# Autodesk Inventor assembly: HDR_2.54mm_RGB4078660
(part 2 of 3)
- D:\Github\Pandoras_Box\CAD\pandoras_box_R2\pandoras_box_R2\Open CASCADE STEP translator 6.8 1.452.1.450.ipt
- D:\Github\Pandoras_Box\CAD\pandoras_box_R2\pandoras_box_R2\Open CASCADE STEP translator 6.8 1.452.1.451.ipt
- D:\Github\Pandoras_Box\CAD\pandoras_box_R2\pandoras_box_R2\Open CASCADE STEP translator 6.8 1.452.1.452.ipt
- D:\Github\Pandoras_Box\CAD\pandoras_box_R2\pandoras_box_R2\Open CASCADE STEP translator 6.8 1.452.1.453.ipt
- D:\Github\Pandoras_Box\CAD\pandoras_box_R2\pandoras_box_R2\Open CASCADE STEP translator 6.8 1.452.1.454.ipt
- D:\Github\Pandoras_Box\CAD\pandoras_box_R2\pandoras_box_R2\Open CASCADE STEP translator 6.8 1.452.1.455.ipt
- D:\Github\Pandoras_Box\CAD\pandoras_box_R2\pandoras_box_R2\Open CASCADE STEP translator 6.8 1.452.1.456.ipt
- D:\Github\Pandoras_Box\CAD\pandoras_box_R2\pandoras_box_R2\Open CASCADE STEP translator 6.8 1.452.1.457.ipt
- D:\Github\Pandoras_Box\CAD\pandoras_box_R2\pandoras_box_R2\Open CASCADE STEP translator 6.8 1.452.1.458.ipt
- D:\Github\Pandoras_Box\CAD\pandoras_box_R2\pandoras_box_R2\Open CASCADE STEP translator 6.8 1.452.1.459.ipt
- D:\Github\Pandoras_Box\CAD\pandoras_box_R2\pandoras_box_R2\Open CASCADE STEP translator 6.8 1.452.1.460.ipt
- D:\Github\Pandoras_Box\CAD\pandoras_box_R2\pandoras_box_R2\Open CASCADE STEP translator 6.8 1.452.1.461.ipt
- D:\Github\Pandoras_Box\CAD\pandoras_box_R2\pandoras_box_R2\Open CASCADE STEP translator 6.8 1.452.1.462.ipt
- D:\Github\Pandoras_Box\CAD\pandoras_box_R2\pandoras_box_R2\Open CASCADE STEP translator 6.8 1.452.1.463.ipt
- D:\Github\Pandoras_Box\CAD\pandoras_box_R2\pandoras_box_R2\Open CASCADE STEP translator 6.8 1.452.1.464.ipt
- D:\Github\Pandoras_Box\CAD\pandoras_box_R2\pandoras_box_R2\Open CASCADE STEP translator 6.8 1.452.1.465.ipt
- D:\Github\Pandoras_Box\CAD\pandoras_box_R2\pandoras_box_R2\Open CASCADE STEP translator 6.8 1.452.1.466.ipt
- D:\Github\Pandoras_Box\CAD\pandoras_box_R2\pandoras_box_R2\Open CASCADE STEP translator 6.8 1.452.1.467.ipt
- D:\Github\Pandoras_Box\CAD\pandoras_box_R2\pandoras_box_R2\Open CASCADE STEP translator 6.8 1.452.1.468.ipt
- D:\Github\Pandoras_Box\CAD\pandoras_box_R2\pandoras_box_R2\Open CASCADE STEP translator 6.8 1.452.1.469.ipt
- D:\Github\Pandoras_Box\CAD\pandoras_box_R2\pandoras_box_R2\Open CASCADE STEP translator 6.8 1.452.1.470.ipt
- D:\Github\Pandoras_Box\CAD\pandoras_box_R2\pandoras_box_R2\Open CASCADE STEP translator 6.8 1.452.1.471.ipt
- D:\Github\Pandoras_Box\CAD\pandoras_box_R2\pandoras_box_R2\Open CASCADE STEP translator 6.8 1.452.1.472.ipt
- D:\Github\Pandoras_Box\CAD\pandoras_box_R2\pandoras_box_R2\Open CASCADE STEP translator 6.8 1.452.1.473.ipt
- D:\Github\Pandoras_Box\CAD\pandoras_box_R2\pandoras_box_R2\Open CASCADE STEP translator 6.8 1.452.1.474.ipt
- D:\Github\Pandoras_Box\CAD\pandoras_box_R2\pandoras_box_R2\Open CASCADE STEP translator 6.8 1.452.1.475.ipt
- D:\Github\Pandoras_Box\CAD\pandoras_box_R2\pandoras_box_R2\Open CASCADE STEP translator 6.8 1.452.1.476.ipt
- D:\Github\Pandoras_Box\CAD\pandoras_box_R2\pandoras_box_R2\Open CASCADE STEP translator 6.8 1.452.1.477.ipt
- D:\Github\Pandoras_Box\CAD\pandoras_box_R2\pandoras_box_R2\Open CASCADE STEP translator 6.8 1.452.1.478.ipt
- D:\Github\Pandoras_Box\CAD\pandoras_box_R2\pandoras_box_R2\Open CASCADE STEP translator 6.8 1.452.1.479.ipt
- D:\Github\Pandoras_Box\CAD\pandoras_box_R2\pandoras_box_R2\Open CASCADE STEP translator 6.8 1.452.1.480.ipt
- D:\Github\Pandoras_Box\CAD\pandoras_box_R2\pandoras_box_R2\Open CASCADE STEP translator 6.8 1.452.1.481.ipt
- D:\Github\Pandoras_Box\CAD\pandoras_box_R2\pandoras_box_R2\Open CASCADE STEP translator 6.8 1.452.1.482.ipt
- D:\Github\Pandoras_Box\CAD\pandoras_box_R2\pandoras_box_R2\Open CASCADE STEP translator 6.8 1.452.1.483.ipt
- D:\Github\Pandoras_Box\CAD\pandoras_box_R2\pandoras_box_R2\Open CASCADE STEP translator 6.8 1.452.1.484.ipt
- D:\Github\Pandoras_Box\CAD\pandoras_box_R2\pandoras_box_R2\Open CASCADE STEP translator 6.8 1.452.1.485.ipt
- D:\Github\Pandoras_Box\CAD\pandoras_box_R2\pandoras_box_R2\Open CASCADE STEP translator 6.8 1.452.1.486.ipt
- D:\Github\Pandoras_Box\CAD\pandoras_box_R2\pandoras_box_R2\Open CASCADE STEP translator 6.8 1.452.1.487.ipt
- D:\Github\Pandoras_Box\CAD\pandoras_box_R2\pandoras_box_R2\Open CASCADE STEP translator 6.8 1.452.1.488.ipt
- D:\Github\Pandoras_Box\CAD\pandoras_box_R2\pandoras_box_R2\Open CASCADE STEP translator 6.8 1.452.1.489.ipt
- D:\Github\Pandoras_Box\CAD\pandoras_box_R2\pandoras_box_R2\Open CASCADE STEP translator 6.8 1.452.1.490.ipt
- D:\Github\Pandoras_Box\CAD\pandoras_box_R2\pandoras_box_R2\Open CASCADE STEP translator 6.8 1.452.1.491.ipt
- D:\Github\Pandoras_Box\CAD\pandoras_box_R2\pandoras_box_R2\Open CASCADE STEP translator 6.8 1.452.1.492.ipt
- D:\Github\Pandoras_Box\CAD\pandoras_box_R2\pandoras_box_R2\Open CASCADE STEP translator 6.8 1.452.1.493.ipt
- D:\Github\Pandoras_Box\CAD\pandoras_box_R2\pandoras_box_R2\Open CASCADE STEP translator 6.8 1.452.1.494.ipt
- D:\Github\Pandoras_Box\CAD\pandoras_box_R2\pandoras_box_R2\Open CASCADE STEP translator 6.8 1.452.1.495.ipt
- D:\Github\Pandoras_Box\CAD\pandoras_box_R2\pandoras_box_R2\Open CASCADE STEP translator 6.8 1.452.1.496.ipt
- D:\Github\Pandoras_Box\CAD\pandoras_box_R2\pandoras_box_R2\Open CASCADE STEP translator 6.8 1.452.1.497.ipt
- D:\Github\Pandoras_Box\CAD\pandoras_box_R2\pandoras_box_R2\Open CASCADE STEP translator 6.8 1.452.1.498.ipt
- D:\Github\Pandoras_Box\CAD\pandoras_box_R2\pandoras_box_R2\Open CASCADE STEP translator 6.8 1.452.1.499.ipt
- D:\Github\Pandoras_Box\CAD\pandoras_box_R2\pandoras_box_R2\Open CASCADE STEP translator 6.8 1.452.1.500.ipt
- D:\Github\Pandoras_Box\CAD\pandoras_box_R2\pandoras_box_R2\Open CASCADE STEP translator 6.8 1.452.1.501.ipt
- D:\Github\Pandoras_Box\CAD\pandoras_box_R2\pandoras_box_R2\Open CASCADE STEP translator 6.8 1.452.1.502.ipt
- D:\Github\Pandoras_Box\CAD\pandoras_box_R2\pandoras_box_R2\Open CASCADE STEP translator 6.8 1.452.1.503.ipt
- D:\Github\Pandoras_Box\CAD\pandoras_box_R2\pandoras_box_R2\Open CASCADE STEP translator 6.8 1.452.1.504.ipt
- D:\Github\Pandoras_Box\CAD\pandoras_box_R2\pandoras_box_R2\Open CASCADE STEP translator 6.8 1.452.1.505.ipt
- D:\Github\Pandoras_Box\CAD\pandoras_box_R2\pandoras_box_R2\Open CASCADE STEP translator 6.8 1.452.1.506.ipt
- D:\Github\Pandoras_Box\CAD\pandoras_box_R2\pandoras_box_R2\Open CASCADE STEP translator 6.8 1.452.1.507.ipt
- D:\Github\Pandoras_Box\CAD\pandoras_box_R2\pandoras_box_R2\Open CASCADE STEP translator 6.8 1.452.1.508.ipt
- D:\Github\Pandoras_Box\CAD\pandoras_box_R2\pandoras_box_R2\Open CASCADE STEP translator 6.8 1.452.1.509.ipt
- D:\Github\Pandoras_Box\CAD\pandoras_box_R2\pandoras_box_R2\Open CASCADE STEP translator 6.8 1.452.1.510.ipt
- D:\Github\Pandoras_Box\CAD\pandoras_box_R2\pandoras_box_R2\Open CASCADE STEP translator 6.8 1.452.1.511.ipt
- D:\Github\Pandoras_Box\CAD\pandoras_box_R2\pandoras_box_R2\Open CASCADE STEP translator 6.8 1.452.1.512.ipt
- D:\Github\Pandoras_Box\CAD\pandoras_box_R2\pandoras_box_R2\Open CASCADE STEP translator 6.8 1.452.1.513.ipt
- D:\Github\Pandoras_Box\CAD\pandoras_box_R2\pandoras_box_R2\Open CASCADE STEP translator 6.8 1.452.1.514.ipt
- D:\Github\Pandoras_Box\CAD\pandoras_box_R2\pandoras_box_R2\Open CASCADE STEP translator 6.8 1.452.1.515.ipt
- D:\Github\Pandoras_Box\CAD\pandoras_box_R2\pandoras_box_R2\Open CASCADE STEP translator 6.8 1.452.1.516.ipt
- D:\Github\Pandoras_Box\CAD\pandoras_box_R2\pandoras_box_R2\Open CASCADE STEP translator 6.8 1.452.1.517.ipt
- D:\Github\Pandoras_Box\CAD\pandoras_box_R2\pandoras_box_R2\Open CASCADE STEP translator 6.8 1.452.1.518.ipt
- D:\Github\Pandoras_Box\CAD\pandoras_box_R2\pandoras_box_R2\Open CASCADE STEP translator 6.8 1.452.1.519.ipt
- D:\Github\Pandoras_Box\CAD\pandoras_box_R2\pandoras_box_R2\Open CASCADE STEP translator 6.8 1.452.1.520.ipt
- D:\Github\Pandoras_Box\CAD\pandoras_box_R2\pandoras_box_R2\Open CASCADE STEP translator 6.8 1.452.1.521.ipt
- D:\Github\Pandoras_Box\CAD\pandoras_box_R2\pandoras_box_R2\Open CASCADE STEP translator 6.8 1.452.1.522.ipt
- D:\Github\Pandoras_Box\CAD\pandoras_box_R2\pandoras_box_R2\Open CASCADE STEP translator 6.8 1.452.1.523.ipt
- D:\Github\Pandoras_Box\CAD\pandoras_box_R2\pandoras_box_R2\Open CASCADE STEP translator 6.8 1.452.1.524.ipt
- D:\Github\Pandoras_Box\CAD\pandoras_box_R2\pandoras_box_R2\Open CASCADE STEP translator 6.8 1.452.1.525.ipt
- D:\Github\Pandoras_Box\CAD\pandoras_box_R2\pandoras_box_R2\Open CASCADE STEP translator 6.8 1.452.1.526.ipt
- D:\Github\Pandoras_Box\CAD\pandoras_box_R2\pandoras_box_R2\Open CASCADE STEP translator 6.8 1.452.1.527.ipt
- D:\Github\Pandoras_Box\CAD\pandoras_box_R2\pandoras_box_R2\Open CASCADE STEP translator 6.8 1.452.1.528.ipt
- D:\Github\Pandoras_Box\CAD\pandoras_box_R2\pandoras_box_R2\Open CASCADE STEP translator 6.8 1.452.1.529.ipt
- D:\Github\Pandoras_Box\CAD\pandoras_box_R2\pandoras_box_R2\Open CASCADE STEP translator 6.8 1.452.1.530.ipt
- D:\Github\Pandoras_Box\CAD\pandoras_box_R2\pandoras_box_R2\Open CASCADE STEP translator 6.8 1.452.1.531.ipt
- D:\Github\Pandoras_Box\CAD\pandoras_box_R2\pandoras_box_R2\Open CASCADE STEP translator 6.8 1.452.1.532.ipt
- D:\Github\Pandoras_Box\CAD\pandoras_box_R2\pandoras_box_R2\Open CASCADE STEP translator 6.8 1.452.1.533.ipt
- D:\Github\Pandoras_Box\CAD\pandoras_box_R2\pandoras_box_R2\Open CASCADE STEP translator 6.8 1.452.1.534.ipt
- D:\Github\Pandoras_Box\CAD\pandoras_box_R2\pandoras_box_R2\Open CASCADE STEP translator 6.8 1.452.1.535.ipt
- D:\Github\Pandoras_Box\CAD\pandoras_box_R2\pandoras_box_R2\Open CASCADE STEP translator 6.8 1.452.1.536.ipt
- D:\Github\Pandoras_Box\CAD\pandoras_box_R2\pandoras_box_R2\Open CASCADE STEP translator 6.8 1.452.1.537.ipt
- D:\Github\Pandoras_Box\CAD\pandoras_box_R2\pandoras_box_R2\Open CASCADE STEP translator 6.8 1.452.1.538.ipt
- D:\Github\Pandoras_Box\CAD\pandoras_box_R2\pandoras_box_R2\Open CASCADE STEP translator 6.8 1.452.1.539.ipt
- D:\Github\Pandoras_Box\CAD\pandoras_box_R2\pandoras_box_R2\Open CASCADE STEP translator 6.8 1.452.1.540.ipt
- D:\Github\Pandoras_Box\CAD\pandoras_box_R2\pandoras_box_R2\Open CASCADE STEP translator 6.8 1.452.1.541.ipt
- D:\Github\Pandoras_Box\CAD\pandoras_box_R2\pandoras_box_R2\Open CASCADE STEP translator 6.8 1.452.1.542.ipt
- D:\Github\Pandoras_Box\CAD\pandoras_box_R2\pandoras_box_R2\Open CASCADE STEP translator 6.8 1.452.1.543.ipt
- D:\Github\Pandoras_Box\CAD\pandoras_box_R2\pandoras_box_R2\Open CASCADE STEP translator 6.8 1.452.1.544.ipt
- D:\Github\Pandoras_Box\CAD\pandoras_box_R2\pandoras_box_R2\Open CASCADE STEP translator 6.8 1.452.1.545.ipt
- D:\Github\Pandoras_Box\CAD\pandoras_box_R2\pandoras_box_R2\Open CASCADE STEP translator 6.8 1.452.1.546.ipt
- D:\Github\Pandoras_Box\CAD\pandoras_box_R2\pandoras_box_R2\Open CASCADE STEP translator 6.8 1.452.1.547.ipt
- D:\Github\Pandoras_Box\CAD\pandoras_box_R2\pandoras_box_R2\Open CASCADE STEP translator 6.8 1.452.1.548.ipt
- D:\Github\Pandoras_Box\CAD\pandoras_box_R2\pandoras_box_R2\Open CASCADE STEP translator 6.8 1.452.1.549.ipt
- D:\Github\Pandoras_Box\CAD\pandoras_box_R2\pandoras_box_R2\Open CASCADE STEP translator 6.8 1.452.1.550.ipt
- D:\Github\Pandoras_Box\CAD\pandoras_box_R2\pandoras_box_R2\Open CASCADE STEP translator 6.8 1.452.1.551.ipt
- D:\Github\Pandoras_Box\CAD\pandoras_box_R2\pandoras_box_R2\Open CASCADE STEP translator 6.8 1.452.1.552.ipt
- D:\Github\Pandoras_Box\CAD\pandoras_box_R2\pandoras_box_R2\Open CASCADE STEP translator 6.8 1.452.1.553.ipt
- D:\Github\Pandoras_Box\CAD\pandoras_box_R2\pandoras_box_R2\Open CASCADE STEP translator 6.8 1.452.1.554.ipt
- D:\Github\Pandoras_Box\CAD\pandoras_box_R2\pandoras_box_R2\Open CASCADE STEP translator 6.8 1.452.1.555.ipt
- D:\Github\Pandoras_Box\CAD\pandoras_box_R2\pandoras_box_R2\Open CASCADE STEP translator 6.8 1.452.1.556.ipt
- D:\Github\Pandoras_Box\CAD\pandoras_box_R2\pandoras_box_R2\Open CASCADE STEP translator 6.8 1.452.1.557.ipt
- D:\Github\Pandoras_Box\CAD\pandoras_box_R2\pandoras_box_R2\Open CASCADE STEP translator 6.8 1.452.1.558.ipt
- D:\Github\Pandoras_Box\CAD\pandoras_box_R2\pandoras_box_R2\Open CASCADE STEP translator 6.8 1.452.1.559.ipt
- D:\Github\Pandoras_Box\CAD\pandoras_box_R2\pandoras_box_R2\Open CASCADE STEP translator 6.8 1.452.1.560.ipt
- D:\Github\Pandoras_Box\CAD\pandoras_box_R2\pandoras_box_R2\Open CASCADE STEP translator 6.8 1.452.1.561.ipt
- D:\Github\Pandoras_Box\CAD\pandoras_box_R2\pandoras_box_R2\Open CASCADE STEP translator 6.8 1.452.1.562.ipt
- D:\Github\Pandoras_Box\CAD\pandoras_box_R2\pandoras_box_R2\Open CASCADE STEP translator 6.8 1.452.1.563.ipt
- D:\Github\Pandoras_Box\CAD\pandoras_box_R2\pandoras_box_R2\Open CASCADE STEP translator 6.8 1.452.1.564.ipt
- D:\Github\Pandoras_Box\CAD\pandoras_box_R2\pandoras_box_R2\Open CASCADE STEP translator 6.8 1.452.1.565.ipt
- D:\Github\Pandoras_Box\CAD\pandoras_box_R2\pandoras_box_R2\Open CASCADE STEP translator 6.8 1.452.1.566.ipt
- D:\Github\Pandoras_Box\CAD\pandoras_box_R2\pandoras_box_R2\Open CASCADE STEP translator 6.8 1.452.1.567.ipt
- D:\Github\Pandoras_Box\CAD\pandoras_box_R2\pandoras_box_R2\Open CASCADE STEP translator 6.8 1.452.1.568.ipt
- D:\Github\Pandoras_Box\CAD\pandoras_box_R2\pandoras_box_R2\Open CASCADE STEP translator 6.8 1.452.1.569.ipt
- D:\Github\Pandoras_Box\CAD\pandoras_box_R2\pandoras_box_R2\Open CASCADE STEP translator 6.8 1.452.1.570.ipt
- D:\Github\Pandoras_Box\CAD\pandoras_box_R2\pandoras_box_R2\Open CASCADE STEP translator 6.8 1.452.1.571.ipt
- D:\Github\Pandoras_Box\CAD\pandoras_box_R2\pandoras_box_R2\Open CASCADE STEP translator 6.8 1.452.1.572.ipt
- D:\Github\Pandoras_Box\CAD\pandoras_box_R2\pandoras_box_R2\Open CASCADE STEP translator 6.8 1.452.1.573.ipt
- D:\Github\Pandoras_Box\CAD\pandoras_box_R2\pandoras_box_R2\Open CASCADE STEP translator 6.8 1.452.1.574.ipt
- D:\Github\Pandoras_Box\CAD\pandoras_box_R2\pandoras_box_R2\Open CASCADE STEP translator 6.8 1.452.1.575.ipt
- D:\Github\Pandoras_Box\CAD\pandoras_box_R2\pandoras_box_R2\Open CASCADE STEP translator 6.8 1.452.1.576.ipt
- D:\Github\Pandoras_Box\CAD\pandoras_box_R2\pandoras_box_R2\Open CASCADE STEP translator 6.8 1.452.1.577.ipt
- D:\Github\Pandoras_Box\CAD\pandoras_box_R2\pandoras_box_R2\Open CASCADE STEP translator 6.8 1.452.1.578.ipt
- D:\Github\Pandoras_Box\CAD\pandoras_box_R2\pandoras_box_R2\Open CASCADE STEP translator 6.8 1.452.1.579.ipt
- D:\Github\Pandoras_Box\CAD\pandoras_box_R2\pandoras_box_R2\Open CASCADE STEP translator 6.8 1.452.1.580.ipt
- D:\Github\Pandoras_Box\CAD\pandoras_box_R2\pandoras_box_R2\Open CASCADE STEP translator 6.8 1.452.1.581.ipt
- D:\Github\Pandoras_Box\CAD\pandoras_box_R2\pandoras_box_R2\Open CASCADE STEP translator 6.8 1.452.1.582.ipt
- D:\Github\Pandoras_Box\CAD\pandoras_box_R2\pandoras_box_R2\Open CASCADE STEP translator 6.8 1.452.1.583.ipt
- D:\Github\Pandoras_Box\CAD\pandoras_box_R2\pandoras_box_R2\Open CASCADE STEP translator 6.8 1.452.1.584.ipt
- D:\Github\Pandoras_Box\CAD\pandoras_box_R2\pandoras_box_R2\Open CASCADE STEP translator 6.8 1.452.1.585.ipt
- D:\Github\Pandoras_Box\CAD\pandoras_box_R2\pandoras_box_R2\Open CASCADE STEP translator 6.8 1.452.1.586.ipt
- D:\Github\Pandoras_Box\CAD\pandoras_box_R2\pandoras_box_R2\Open CASCADE STEP translator 6.8 1.452.1.587.ipt
- D:\Github\Pandoras_Box\CAD\pandoras_box_R2\pandoras_box_R2\Open CASCADE STEP translator 6.8 1.452.1.588.ipt
- D:\Github\Pandoras_Box\CAD\pandoras_box_R2\pandoras_box_R2\Open CASCADE STEP translator 6.8 1.452.1.589.ipt
- D:\Github\Pandoras_Box\CAD\pandoras_box_R2\pandoras_box_R2\Open CASCADE STEP translator 6.8 1.452.1.590.ipt
- D:\Github\Pandoras_Box\CAD\pandoras_box_R2\pandoras_box_R2\Open CASCADE STEP translator 6.8 1.452.1.591.ipt
- D:\Github\Pandoras_Box\CAD\pandoras_box_R2\pandoras_box_R2\Open CASCADE STEP translator 6.8 1.452.1.592.ipt
- D:\Github\Pandoras_Box\CAD\pandoras_box_R2\pandoras_box_R2\Open CASCADE STEP translator 6.8 1.452.1.593.ipt
- D:\Github\Pandoras_Box\CAD\pandoras_box_R2\pandoras_box_R2\Open CASCADE STEP translator 6.8 1.452.1.594.ipt
- D:\Github\Pandoras_Box\CAD\pandoras_box_R2\pandoras_box_R2\Open CASCADE STEP translator 6.8 1.452.1.595.ipt
- D:\Github\Pandoras_Box\CAD\pandoras_box_R2\pandoras_box_R2\Open CASCADE STEP translator 6.8 1.452.1.596.ipt
- D:\Github\Pandoras_Box\CAD\pandoras_box_R2\pandoras_box_R2\Open CASCADE STEP translator 6.8 1.452.1.597.ipt
- D:\Github\Pandoras_Box\CAD\pandoras_box_R2\pandoras_box_R2\Open CASCADE STEP translator 6.8 1.452.1.598.ipt
- D:\Github\Pandoras_Box\CAD\pandoras_box_R2\pandoras_box_R2\Open CASCADE STEP translator 6.8 1.452.1.599.ipt
- D:\Github\Pandoras_Box\CAD\pandoras_box_R2\pandoras_box_R2\Open CASCADE STEP translator 6.8 1.452.1.600.ipt
- D:\Github\Pandoras_Box\CAD\pandoras_box_R2\pandoras_box_R2\Open CASCADE STEP translator 6.8 1.452.1.601.ipt
- D:\Github\Pandoras_Box\CAD\pandoras_box_R2\pandoras_box_R2\Open CASCADE STEP translator 6.8 1.452.1.602.ipt
- D:\Github\Pandoras_Box\CAD\pandoras_box_R2\pandoras_box_R2\Open CASCADE STEP translator 6.8 1.452.1.603.ipt
- D:\Github\Pandoras_Box\CAD\pandoras_box_R2\pandoras_box_R2\Open CASCADE STEP translator 6.8 1.452.1.604.ipt
- D:\Github\Pandoras_Box\CAD\pandoras_box_R2\pandoras_box_R2\Open CASCADE STEP translator 6.8 1.452.1.605.ipt
- D:\Github\Pandoras_Box\CAD\pandoras_box_R2\pandoras_box_R2\Open CASCADE STEP translator 6.8 1.452.1.606.ipt
- D:\Github\Pandoras_Box\CAD\pandoras_box_R2\pandoras_box_R2\Open CASCADE STEP translator 6.8 1.452.1.607.ipt
- D:\Github\Pandoras_Box\CAD\pandoras_box_R2\pandoras_box_R2\Open CASCADE STEP translator 6.8 1.452.1.608.ipt
- D:\Github\Pandoras_Box\CAD\pandoras_box_R2\pandoras_box_R2\Open CASCADE STEP translator 6.8 1.452.1.609.ipt
- D:\Github\Pandoras_Box\CAD\pandoras_box_R2\pandoras_box_R2\Open CASCADE STEP translator 6.8 1.452.1.610.ipt
- D:\Github\Pandoras_Box\CAD\pandoras_box_R2\pandoras_box_R2\Open CASCADE STEP translator 6.8 1.452.1.611.ipt
- D:\Github\Pandoras_Box\CAD\pandoras_box_R2\pandoras_box_R2\Open CASCADE STEP translator 6.8 1.452.1.612.ipt
- D:\Github\Pandoras_Box\CAD\pandoras_box_R2\pandoras_box_R2\Open CASCADE STEP translator 6.8 1.452.1.613.ipt
- D:\Github\Pandoras_Box\CAD\pandoras_box_R2\pandoras_box_R2\Open CASCADE STEP translator 6.8 1.452.1.614.ipt
- D:\Github\Pandoras_Box\CAD\pandoras_box_R2\pandoras_box_R2\Open CASCADE STEP translator 6.8 1.452.1.615.ipt
- D:\Github\Pandoras_Box\CAD\pandoras_box_R2\pandoras_box_R2\Open CASCADE STEP translator 6.8 1.452.1.616.ipt
- D:\Github\Pandoras_Box\CAD\pandoras_box_R2\pandoras_box_R2\Open CASCADE STEP translator 6.8 1.452.1.617.ipt
- D:\Github\Pandoras_Box\CAD\pandoras_box_R2\pandoras_box_R2\Open CASCADE STEP translator 6.8 1.452.1.618.ipt
- D:\Github\Pandoras_Box\CAD\pandoras_box_R2\pandoras_box_R2\Open CASCADE STEP translator 6.8 1.452.1.619.ipt
- D:\Github\Pandoras_Box\CAD\pandoras_box_R2\pandoras_box_R2\Open CASCADE STEP translator 6.8 1.452.1.620.ipt
- D:\Github\Pandoras_Box\CAD\pandoras_box_R2\pandoras_box_R2\Open CASCADE STEP translator 6.8 1.452.1.621.ipt
- D:\Github\Pandoras_Box\CAD\pandoras_box_R2\pandoras_box_R2\Open CASCADE STEP translator 6.8 1.452.1.622.ipt
- D:\Github\Pandoras_Box\CAD\pandoras_box_R2\pandoras_box_R2\Open CASCADE STEP translator 6.8 1.452.1.623.ipt
- D:\Github\Pandoras_Box\CAD\pandoras_box_R2\pandoras_box_R2\Open CASCADE STEP translator 6.8 1.452.1.624.ipt
## Components (624 placed, 624 different names)
1. Open CASCADE STEP translator 6.8 1.452.1.1:1
2. Open CASCADE STEP translator 6.8 1.452.1.2:1
3. Open CASCADE STEP translator 6.8 1.452.1.3:1
4. Open CASCADE STEP translator 6.8 1.452.1.4:1
5. Open CASCADE STEP translator 6.8 1.452.1.5:1
6. Open CASCADE STEP translator 6.8 1.452.1.6:1
7. Open CASCADE STEP translator 6.8 1.452.1.7:1
8. Open CASCADE STEP translator 6.8 1.452.1.8:1
9. Open CASCADE STEP translator 6.8 1.452.1.9:1
10. Open CASCADE STEP translator 6.8 1.452.1.10:1
11. Open CASCADE STEP translator 6.8 1.452.1.11:1
12. Open CASCADE STEP translator 6.8 1.452.1.12:1
13. Open CASCADE STEP translator 6.8 1.452.1.13:1
14. Open CASCADE STEP translator 6.8 1.452.1.14:1
15. Open CASCADE STEP translator 6.8 1.452.1.15:1
16. Open CASCADE STEP translator 6.8 1.452.1.16:1
17. Open CASCADE STEP translator 6.8 1.452.1.17:1
18. Open CASCADE STEP translator 6.8 1.452.1.18:1
19. Open CASCADE STEP translator 6.8 1.452.1.19:1
20. Open CASCADE STEP translator 6.8 1.452.1.20:1
21. Open CASCADE STEP translator 6.8 1.452.1.21:1
22. Open CASCADE STEP translator 6.8 1.452.1.22:1
23. Open CASCADE STEP translator 6.8 1.452.1.23:1
24. Open CASCADE STEP translator 6.8 1.452.1.24:1
25. Open CASCADE STEP translator 6.8 1.452.1.25:1
26. Open CASCADE STEP translator 6.8 1.452.1.26:1
27. Open CASCADE STEP translator 6.8 1.452.1.27:1
28. Open CASCADE STEP translator 6.8 1.452.1.28:1
29. Open CASCADE STEP translator 6.8 1.452.1.29:1
30. Open CASCADE STEP translator 6.8 1.452.1.30:1
31. Open CASCADE STEP translator 6.8 1.452.1.31:1
32. Open CASCADE STEP translator 6.8 1.452.1.32:1
33. Open CASCADE STEP translator 6.8 1.452.1.33:1
34. Open CASCADE STEP translator 6.8 1.452.1.34:1
35. Open CASCADE STEP translator 6.8 1.452.1.35:1
36. Open CASCADE STEP translator 6.8 1.452.1.36:1
37. Open CASCADE STEP translator 6.8 1.452.1.37:1
38. Open CASCADE STEP translator 6.8 1.452.1.38:1
39. Open CASCADE STEP translator 6.8 1.452.1.39:1
40. Open CASCADE STEP translator 6.8 1.452.1.40:1
41. Open CASCADE STEP translator 6.8 1.452.1.41:1
42. Open CASCADE STEP translator 6.8 1.452.1.42:1
43. Open CASCADE STEP translator 6.8 1.452.1.43:1
44. Open CASCADE STEP translator 6.8 1.452.1.44:1
45. Open CASCADE STEP translator 6.8 1.452.1.45:1
46. Open CASCADE STEP translator 6.8 1.452.1.46:1
47. Open CASCADE STEP translator 6.8 1.452.1.47:1
48. Open CASCADE STEP translator 6.8 1.452.1.48:1
49. Open CASCADE STEP translator 6.8 1.452.1.49:1
50. Open CASCADE STEP translator 6.8 1.452.1.50:1
51. Open CASCADE STEP translator 6.8 1.452.1.51:1
52. Open CASCADE STEP translator 6.8 1.452.1.52:1
53. Open CASCADE STEP translator 6.8 1.452.1.53:1
54. Open CASCADE STEP translator 6.8 1.452.1.54:1
55. Open CASCADE STEP translator 6.8 1.452.1.55:1
56. Open CASCADE STEP translator 6.8 1.452.1.56:1
57. Open CASCADE STEP translator 6.8 1.452.1.57:1
58. Open CASCADE STEP translator 6.8 1.452.1.58:1
59. Open CASCADE STEP translator 6.8 1.452.1.59:1
60. Open CASCADE STEP translator 6.8 1.452.1.60:1
61. Open CASCADE STEP translator 6.8 1.452.1.61:1
62. Open CASCADE STEP translator 6.8 1.452.1.62:1
63. Open CASCADE STEP translator 6.8 1.452.1.63:1
64. Open CASCADE STEP translator 6.8 1.452.1.64:1
65. Open CASCADE STEP translator 6.8 1.452.1.65:1
66. Open CASCADE STEP translator 6.8 1.452.1.66:1
67. Open CASCADE STEP translator 6.8 1.452.1.67:1
68. Open CASCADE STEP translator 6.8 1.452.1.68:1
69. Open CASCADE STEP translator 6.8 1.452.1.69:1
70. Open CASCADE STEP translator 6.8 1.452.1.70:1
71. Open CASCADE STEP translator 6.8 1.452.1.71:1
72. Open CASCADE STEP translator 6.8 1.452.1.72:1
73. Open CASCADE STEP translator 6.8 1.452.1.73:1
74. Open CASCADE STEP translator 6.8 1.452.1.74:1
75. Open CASCADE STEP translator 6.8 1.452.1.75:1
76. Open CASCADE STEP translator 6.8 1.452.1.76:1
77. Open CASCADE STEP translator 6.8 1.452.1.77:1
78. Open CASCADE STEP translator 6.8 1.452.1.78:1
79. Open CASCADE STEP translator 6.8 1.452.1.79:1
80. Open CASCADE STEP translator 6.8 1.452.1.80:1
81. Open CASCADE STEP translator 6.8 1.452.1.81:1
82. Open CASCADE STEP translator 6.8 1.452.1.82:1
83. Open CASCADE STEP translator 6.8 1.452.1.83:1
84. Open CASCADE STEP translator 6.8 1.452.1.84:1
85. Open CASCADE STEP translator 6.8 1.452.1.85:1
86. Open CASCADE STEP translator 6.8 1.452.1.86:1
87. Open CASCADE STEP translator 6.8 1.452.1.87:1
88. Open CASCADE STEP translator 6.8 1.452.1.88:1
89. Open CASCADE STEP translator 6.8 1.452.1.89:1
90. Open CASCADE STEP translator 6.8 1.452.1.90:1
91. Open CASCADE STEP translator 6.8 1.452.1.91:1
92. Open CASCADE STEP translator 6.8 1.452.1.92:1
93. Open CASCADE STEP translator 6.8 1.452.1.93:1
94. Open CASCADE STEP translator 6.8 1.452.1.94:1
95. Open CASCADE STEP translator 6.8 1.452.1.95:1
96. Open CASCADE STEP translator 6.8 1.452.1.96:1
97. Open CASCADE STEP translator 6.8 1.452.1.97:1
98. Open CASCADE STEP translator 6.8 1.452.1.98:1
99. Open CASCADE STEP translator 6.8 1.452.1.99:1
100. Open CASCADE STEP translator 6.8 1.452.1.100:1
101. Open CASCADE STEP translator 6.8 1.452.1.101:1
102. Open CASCADE STEP translator 6.8 1.452.1.102:1
103. Open CASCADE STEP translator 6.8 1.452.1.103:1
104. Open CASCADE STEP translator 6.8 1.452.1.104:1
105. Open CASCADE STEP translator 6.8 1.452.1.105:1
106. Open CASCADE STEP translator 6.8 1.452.1.106:1
107. Open CASCADE STEP translator 6.8 1.452.1.107:1
108. Open CASCADE STEP translator 6.8 1.452.1.108:1
109. Open CASCADE STEP translator 6.8 1.452.1.109:1
110. Open CASCADE STEP translator 6.8 1.452.1.110:1
111. Open CASCADE STEP translator 6.8 1.452.1.111:1
112. Open CASCADE STEP translator 6.8 1.452.1.112:1
113. Open CASCADE STEP translator 6.8 1.452.1.113:1
114. Open CASCADE STEP translator 6.8 1.452.1.114:1
115. Open CASCADE STEP translator 6.8 1.452.1.115:1
116. Open CASCADE STEP translator 6.8 1.452.1.116:1
117. Open CASCADE STEP translator 6.8 1.452.1.117:1
118. Open CASCADE STEP translator 6.8 1.452.1.118:1
119. Open CASCADE STEP translator 6.8 1.452.1.119:1
120. Open CASCADE STEP translator 6.8 1.452.1.120:1
121. Open CASCADE STEP translator 6.8 1.452.1.121:1
122. Open CASCADE STEP translator 6.8 1.452.1.122:1
123. Open CASCADE STEP translator 6.8 1.452.1.123:1
124. Open CASCADE STEP translator 6.8 1.452.1.124:1
125. Open CASCADE STEP translator 6.8 1.452.1.125:1
126. Open CASCADE STEP translator 6.8 1.452.1.126:1
127. Open CASCADE STEP translator 6.8 1.452.1.127:1
128. Open CASCADE STEP translator 6.8 1.452.1.128:1
129. Open CASCADE STEP translator 6.8 1.452.1.129:1
130. Open CASCADE STEP translator 6.8 1.452.1.130:1
131. Open CASCADE STEP translator 6.8 1.452.1.131:1
132. Open CASCADE STEP translator 6.8 1.452.1.132:1
133. Open CASCADE STEP translator 6.8 1.452.1.133:1
134. Open CASCADE STEP translator 6.8 1.452.1.134:1
135. Open CASCADE STEP translator 6.8 1.452.1.135:1
136. Open CASCADE STEP translator 6.8 1.452.1.136:1
137. Open CASCADE STEP translator 6.8 1.452.1.137:1
138. Open CASCADE STEP translator 6.8 1.452.1.138:1
139. Open CASCADE STEP translator 6.8 1.452.1.139:1
140. Open CASCADE STEP translator 6.8 1.452.1.140:1
141. Open CASCADE STEP translator 6.8 1.452.1.141:1
142. Open CASCADE STEP translator 6.8 1.452.1.142:1
143. Open CASCADE STEP translator 6.8 1.452.1.143:1
144. Open CASCADE STEP translator 6.8 1.452.1.144:1
145. Open CASCADE STEP translator 6.8 1.452.1.145:1
146. Open CASCADE STEP translator 6.8 1.452.1.146:1
147. Open CASCADE STEP translator 6.8 1.452.1.147:1
148. Open CASCADE STEP translator 6.8 1.452.1.148:1
149. Open CASCADE STEP translator 6.8 1.452.1.149:1
150. Open CASCADE STEP translator 6.8 1.452.1.150:1
151. Open CASCADE STEP translator 6.8 1.452.1.151:1
152. Open CASCADE STEP translator 6.8 1.452.1.152:1
153. Open CASCADE STEP translator 6.8 1.452.1.153:1
154. Open CASCADE STEP translator 6.8 1.452.1.154:1
155. Open CASCADE STEP translator 6.8 1.452.1.155:1
156. Open CASCADE STEP translator 6.8 1.452.1.156:1
157. Open CASCADE STEP translator 6.8 1.452.1.157:1
158. Open CASCADE STEP translator 6.8 1.452.1.158:1
159. Open CASCADE STEP translator 6.8 1.452.1.159:1
160. Open CASCADE STEP translator 6.8 1.452.1.160:1
161. Open CASCADE STEP translator 6.8 1.452.1.161:1
162. Open CASCADE STEP translator 6.8 1.452.1.162:1
163. Open CASCADE STEP translator 6.8 1.452.1.163:1
164. Open CASCADE STEP translator 6.8 1.452.1.164:1
165. Open CASCADE STEP translator 6.8 1.452.1.165:1
166. Open CASCADE STEP translator 6.8 1.452.1.166:1
167. Open CASCADE STEP translator 6.8 1.452.1.167:1
168. Open CASCADE STEP translator 6.8 1.452.1.168:1
169. Open CASCADE STEP translator 6.8 1.452.1.169:1
170. Open CASCADE STEP translator 6.8 1.452.1.170:1
171. Open CASCADE STEP translator 6.8 1.452.1.171:1
172. Open CASCADE STEP translator 6.8 1.452.1.172:1
173. Open CASCADE STEP translator 6.8 1.452.1.173:1
174. Open CASCADE STEP translator 6.8 1.452.1.174:1
175. Open CASCADE STEP translator 6.8 1.452.1.175:1
176. Open CASCADE STEP translator 6.8 1.452.1.176:1
177. Open CASCADE STEP translator 6.8 1.452.1.177:1
178. Open CASCADE STEP translator 6.8 1.452.1.178:1
179. Open CASCADE STEP translator 6.8 1.452.1.179:1
180. Open CASCADE STEP translator 6.8 1.452.1.180:1
181. Open CASCADE STEP translator 6.8 1.452.1.181:1
182. Open CASCADE STEP translator 6.8 1.452.1.182:1
183. Open CASCADE STEP translator 6.8 1.452.1.183:1
184. Open CASCADE STEP translator 6.8 1.452.1.184:1
185. Open CASCADE STEP translator 6.8 1.452.1.185:1
186. Open CASCADE STEP translator 6.8 1.452.1.186:1
187. Open CASCADE STEP translator 6.8 1.452.1.187:1
188. Open CASCADE STEP translator 6.8 1.452.1.188:1
189. Open CASCADE STEP translator 6.8 1.452.1.189:1
190. Open CASCADE STEP translator 6.8 1.452.1.190:1
191. Open CASCADE STEP translator 6.8 1.452.1.191:1
192. Open CASCADE STEP translator 6.8 1.452.1.192:1
193. Open CASCADE STEP translator 6.8 1.452.1.193:1
194. Open CASCADE STEP translator 6.8 1.452.1.194:1
195. Open CASCADE STEP translator 6.8 1.452.1.195:1
196. Open CASCADE STEP translator 6.8 1.452.1.196:1
197. Open CASCADE STEP translator 6.8 1.452.1.197:1
198. Open CASCADE STEP translator 6.8 1.452.1.198:1
199. Open CASCADE STEP translator 6.8 1.452.1.199:1
200. Open CASCADE STEP translator 6.8 1.452.1.200:1
201. Open CASCADE STEP translator 6.8 1.452.1.201:1
202. Open CASCADE STEP translator 6.8 1.452.1.202:1
203. Open CASCADE STEP translator 6.8 1.452.1.203:1
204. Open CASCADE STEP translator 6.8 1.452.1.204:1
205. Open CASCADE STEP translator 6.8 1.452.1.205:1
206. Open CASCADE STEP translator 6.8 1.452.1.206:1
207. Open CASCADE STEP translator 6.8 1.452.1.207:1
208. Open CASCADE STEP translator 6.8 1.452.1.208:1
209. Open CASCADE STEP translator 6.8 1.452.1.209:1
210. Open CASCADE STEP translator 6.8 1.452.1.210:1
211. Open CASCADE STEP translator 6.8 1.452.1.211:1
212. Open CASCADE STEP translator 6.8 1.452.1.212:1
213. Open CASCADE STEP translator 6.8 1.452.1.213:1
214. Open CASCADE STEP translator 6.8 1.452.1.214:1
215. Open CASCADE STEP translator 6.8 1.452.1.215:1
216. Open CASCADE STEP translator 6.8 1.452.1.216:1
217. Open CASCADE STEP translator 6.8 1.452.1.217:1
218. Open CASCADE STEP translator 6.8 1.452.1.218:1
219. Open CASCADE STEP translator 6.8 1.452.1.219:1
220. Open CASCADE STEP translator 6.8 1.452.1.220:1
221. Open CASCADE STEP translator 6.8 1.452.1.221:1
222. Open CASCADE STEP translator 6.8 1.452.1.222:1
223. Open CASCADE STEP translator 6.8 1.452.1.223:1
224. Open CASCADE STEP translator 6.8 1.452.1.224:1
225. Open CASCADE STEP translator 6.8 1.452.1.225:1
226. Open CASCADE STEP translator 6.8 1.452.1.226:1
227. Open CASCADE STEP translator 6.8 1.452.1.227:1
228. Open CASCADE STEP translator 6.8 1.452.1.228:1
229. Open CASCADE STEP translator 6.8 1.452.1.229:1
230. Open CASCADE STEP translator 6.8 1.452.1.230:1
231. Open CASCADE STEP translator 6.8 1.452.1.231:1
232. Open CASCADE STEP translator 6.8 1.452.1.232:1
233. Open CASCADE STEP translator 6.8 1.452.1.233:1
234. Open CASCADE STEP translator 6.8 1.452.1.234:1
235. Open CASCADE STEP translator 6.8 1.452.1.235:1
236. Open CASCADE STEP translator 6.8 1.452.1.236:1
237. Open CASCADE STEP translator 6.8 1.452.1.237:1
238. Open CASCADE STEP translator 6.8 1.452.1.238:1
239. Open CASCADE STEP translator 6.8 1.452.1.239:1
240. Open CASCADE STEP translator 6.8 1.452.1.240:1
241. Open CASCADE STEP translator 6.8 1.452.1.241:1
242. Open CASCADE STEP translator 6.8 1.452.1.242:1
243. Open CASCADE STEP translator 6.8 1.452.1.243:1
244. Open CASCADE STEP translator 6.8 1.452.1.244:1
245. Open CASCADE STEP translator 6.8 1.452.1.245:1
246. Open CASCADE STEP translator 6.8 1.452.1.246:1
247. Open CASCADE STEP translator 6.8 1.452.1.247:1
248. Open CASCADE STEP translator 6.8 1.452.1.248:1
249. Open CASCADE STEP translator 6.8 1.452.1.249:1
250. Open CASCADE STEP translator 6.8 1.452.1.250:1
251. Open CASCADE STEP translator 6.8 1.452.1.251:1
252. Open CASCADE STEP translator 6.8 1.452.1.252:1
253. Open CASCADE STEP translator 6.8 1.452.1.253:1
254. Open CASCADE STEP translator 6.8 1.452.1.254:1
255. Open CASCADE STEP translator 6.8 1.452.1.255:1
256. Open CASCADE STEP translator 6.8 1.452.1.256:1
257. Open CASCADE STEP translator 6.8 1.452.1.257:1
258. Open CASCADE STEP translator 6.8 1.452.1.258:1
259. Open CASCADE STEP translator 6.8 1.452.1.259:1
260. Open CASCADE STEP translator 6.8 1.452.1.260:1
261. Open CASCADE STEP translator 6.8 1.452.1.261:1
262. Open CASCADE STEP translator 6.8 1.452.1.262:1
263. Open CASCADE STEP translator 6.8 1.452.1.263:1
264. Open CASCADE STEP translator 6.8 1.452.1.264:1
265. Open CASCADE STEP translator 6.8 1.452.1.265:1
266. Open CASCADE STEP translator 6.8 1.452.1.266:1
267. Open CASCADE STEP translator 6.8 1.452.1.267:1
268. Open CASCADE STEP translator 6.8 1.452.1.268:1
269. Open CASCADE STEP translator 6.8 1.452.1.269:1
270. Open CASCADE STEP translator 6.8 1.452.1.270:1
271. Open CASCADE STEP translator 6.8 1.452.1.271:1
272. Open CASCADE STEP translator 6.8 1.452.1.272:1
273. Open CASCADE STEP translator 6.8 1.452.1.273:1
274. Open CASCADE STEP translator 6.8 1.452.1.274:1
275. Open CASCADE STEP translator 6.8 1.452.1.275:1
276. Open CASCADE STEP translator 6.8 1.452.1.276:1
277. Open CASCADE STEP translator 6.8 1.452.1.277:1
278. Open CASCADE STEP translator 6.8 1.452.1.278:1
279. Open CASCADE STEP translator 6.8 1.452.1.279:1
280. Open CASCADE STEP translator 6.8 1.452.1.280:1
281. Open CASCADE STEP translator 6.8 1.452.1.281:1
282. Open CASCADE STEP translator 6.8 1.452.1.282:1
283. Open CASCADE STEP translator 6.8 1.452.1.283:1
284. Open CASCADE STEP translator 6.8 1.452.1.284:1
285. Open CASCADE STEP translator 6.8 1.452.1.285:1
286. Open CASCADE STEP translator 6.8 1.452.1.286:1
287. Open CASCADE STEP translator 6.8 1.452.1.287:1
288. Open CASCADE STEP translator 6.8 1.452.1.288:1
289. Open CASCADE STEP translator 6.8 1.452.1.289:1
290. Open CASCADE STEP translator 6.8 1.452.1.290:1
291. Open CASCADE STEP translator 6.8 1.452.1.291:1
292. Open CASCADE STEP translator 6.8 1.452.1.292:1
293. Open CASCADE STEP translator 6.8 1.452.1.293:1
294. Open CASCADE STEP translator 6.8 1.452.1.294:1
295. Open CASCADE STEP translator 6.8 1.452.1.295:1
296. Open CASCADE STEP translator 6.8 1.452.1.296:1
297. Open CASCADE STEP translator 6.8 1.452.1.297:1
298. Open CASCADE STEP translator 6.8 1.452.1.298:1
299. Open CASCADE STEP translator 6.8 1.452.1.299:1
300. Open CASCADE STEP translator 6.8 1.452.1.300:1
301. Open CASCADE STEP translator 6.8 1.452.1.301:1
302. Open CASCADE STEP translator 6.8 1.452.1.302:1
303. Open CASCADE STEP translator 6.8 1.452.1.303:1
304. Open CASCADE STEP translator 6.8 1.452.1.304:1
305. Open CASCADE STEP translator 6.8 1.452.1.305:1
306. Open CASCADE STEP translator 6.8 1.452.1.306:1
307. Open CASCADE STEP translator 6.8 1.452.1.307:1
308. Open CASCADE STEP translator 6.8 1.452.1.308:1
309. Open CASCADE STEP translator 6.8 1.452.1.309:1
310. Open CASCADE STEP translator 6.8 1.452.1.310:1
311. Open CASCADE STEP translator 6.8 1.452.1.311:1
312. Open CASCADE STEP translator 6.8 1.452.1.312:1
313. Open CASCADE STEP translator 6.8 1.452.1.313:1
314. Open CASCADE STEP translator 6.8 1.452.1.314:1
315. Open CASCADE STEP translator 6.8 1.452.1.315:1
316. Open CASCADE STEP translator 6.8 1.452.1.316:1
317. Open CASCADE STEP translator 6.8 1.452.1.317:1
318. Open CASCADE STEP translator 6.8 1.452.1.318:1
319. Open CASCADE STEP translator 6.8 1.452.1.319:1
320. Open CASCADE STEP translator 6.8 1.452.1.320:1
321. Open CASCADE STEP translator 6.8 1.452.1.321:1
322. Open CASCADE STEP translator 6.8 1.452.1.322:1
323. Open CASCADE STEP translator 6.8 1.452.1.323:1
324. Open CASCADE STEP translator 6.8 1.452.1.324:1
325. Open CASCADE STEP translator 6.8 1.452.1.325:1
326. Open CASCADE STEP translator 6.8 1.452.1.326:1
327. Open CASCADE STEP translator 6.8 1.452.1.327:1
328. Open CASCADE STEP translator 6.8 1.452.1.328:1
329. Open CASCADE STEP translator 6.8 1.452.1.329:1
330. Open CASCADE STEP translator 6.8 1.452.1.330:1
331. Open CASCADE STEP translator 6.8 1.452.1.331:1
332. Open CASCADE STEP translator 6.8 1.452.1.332:1
333. Open CASCADE STEP translator 6.8 1.452.1.333:1
334. Open CASCADE STEP translator 6.8 1.452.1.334:1
335. Open CASCADE STEP translator 6.8 1.452.1.335:1
336. Open CASCADE STEP translator 6.8 1.452.1.336:1
337. Open CASCADE STEP translator 6.8 1.452.1.337:1
338. Open CASCADE STEP translator 6.8 1.452.1.338:1
339. Open CASCADE STEP translator 6.8 1.452.1.339:1
340. Open CASCADE STEP translator 6.8 1.452.1.340:1
341. Open CASCADE STEP translator 6.8 1.452.1.341:1
342. Open CASCADE STEP translator 6.8 1.452.1.342:1
343. Open CASCADE STEP translator 6.8 1.452.1.343:1
344. Open CASCADE STEP translator 6.8 1.452.1.344:1
345. Open CASCADE STEP translator 6.8 1.452.1.345:1
346. Open CASCADE STEP translator 6.8 1.452.1.346:1
347. Open CASCADE STEP translator 6.8 1.452.1.347:1
348. Open CASCADE STEP translator 6.8 1.452.1.348:1
349. Open CASCADE STEP translator 6.8 1.452.1.349:1
350. Open CASCADE STEP translator 6.8 1.452.1.350:1
351. Open CASCADE STEP translator 6.8 1.452.1.351:1
352. Open CASCADE STEP translator 6.8 1.452.1.352:1
353. Open CASCADE STEP translator 6.8 1.452.1.353:1
354. Open CASCADE STEP translator 6.8 1.452.1.354:1
355. Open CASCADE STEP translator 6.8 1.452.1.355:1
356. Open CASCADE STEP translator 6.8 1.452.1.356:1
357. Open CASCADE STEP translator 6.8 1.452.1.357:1
358. Open CASCADE STEP translator 6.8 1.452.1.358:1
359. Open CASCADE STEP translator 6.8 1.452.1.359:1
360. Open CASCADE STEP translator 6.8 1.452.1.360:1
361. Open CASCADE STEP translator 6.8 1.452.1.361:1
362. Open CASCADE STEP translator 6.8 1.452.1.362:1
363. Open CASCADE STEP translator 6.8 1.452.1.363:1
364. Open CASCADE STEP translator 6.8 1.452.1.364:1
365. Open CASCADE STEP translator 6.8 1.452.1.365:1
366. Open CASCADE STEP translator 6.8 1.452.1.366:1
367. Open CASCADE STEP translator 6.8 1.452.1.367:1
368. Open CASCADE STEP translator 6.8 1.452.1.368:1
369. Open CASCADE STEP translator 6.8 1.452.1.369:1
370. Open CASCADE STEP translator 6.8 1.452.1.370:1
371. Open CASCADE STEP translator 6.8 1.452.1.371:1
372. Open CASCADE STEP translator 6.8 1.452.1.372:1
373. Open CASCADE STEP translator 6.8 1.452.1.373:1
374. Open CASCADE STEP translator 6.8 1.452.1.374:1
375. Open CASCADE STEP translator 6.8 1.452.1.375:1
376. Open CASCADE STEP translator 6.8 1.452.1.376:1
377. Open CASCADE STEP translator 6.8 1.452.1.377:1
378. Open CASCADE STEP translator 6.8 1.452.1.378:1
379. Open CASCADE STEP translator 6.8 1.452.1.379:1
380. Open CASCADE STEP translator 6.8 1.452.1.380:1
381. Open CASCADE STEP translator 6.8 1.452.1.381:1
382. Open CASCADE STEP translator 6.8 1.452.1.382:1
383. Open CASCADE STEP translator 6.8 1.452.1.383:1
384. Open CASCADE STEP translator 6.8 1.452.1.384:1
385. Open CASCADE STEP translator 6.8 1.452.1.385:1
386. Open CASCADE STEP translator 6.8 1.452.1.386:1
387. Open CASCADE STEP translator 6.8 1.452.1.387:1
388. Open CASCADE STEP translator 6.8 1.452.1.388:1
389. Open CASCADE STEP translator 6.8 1.452.1.389:1
390. Open CASCADE STEP translator 6.8 1.452.1.390:1
391. Open CASCADE STEP translator 6.8 1.452.1.391:1
392. Open CASCADE STEP translator 6.8 1.452.1.392:1
393. Open CASCADE STEP translator 6.8 1.452.1.393:1
394. Open CASCADE STEP translator 6.8 1.452.1.394:1
395. Open CASCADE STEP translator 6.8 1.452.1.395:1
396. Open CASCADE STEP translator 6.8 1.452.1.396:1
397. Open CASCADE STEP translator 6.8 1.452.1.397:1
398. Open CASCADE STEP translator 6.8 1.452.1.398:1
399. Open CASCADE STEP translator 6.8 1.452.1.399:1
400. Open CASCADE STEP translator 6.8 1.452.1.400:1
401. Open CASCADE STEP translator 6.8 1.452.1.401:1
402. Open CASCADE STEP translator 6.8 1.452.1.402:1
403. Open CASCADE STEP translator 6.8 1.452.1.403:1
404. Open CASCADE STEP translator 6.8 1.452.1.404:1
405. Open CASCADE STEP translator 6.8 1.452.1.405:1
406. Open CASCADE STEP translator 6.8 1.452.1.406:1
407. Open CASCADE STEP translator 6.8 1.452.1.407:1
408. Open CASCADE STEP translator 6.8 1.452.1.408:1
409. Open CASCADE STEP translator 6.8 1.452.1.409:1
410. Open CASCADE STEP translator 6.8 1.452.1.410:1
411. Open CASCADE STEP translator 6.8 1.452.1.411:1
412. Open CASCADE STEP translator 6.8 1.452.1.412:1
413. Open CASCADE STEP translator 6.8 1.452.1.413:1
414. Open CASCADE STEP translator 6.8 1.452.1.414:1
415. Open CASCADE STEP translator 6.8 1.452.1.415:1
416. Open CASCADE STEP translator 6.8 1.452.1.416:1
417. Open CASCADE STEP translator 6.8 1.452.1.417:1
418. Open CASCADE STEP translator 6.8 1.452.1.418:1
419. Open CASCADE STEP translator 6.8 1.452.1.419:1
420. Open CASCADE STEP translator 6.8 1.452.1.420:1
421. Open CASCADE STEP translator 6.8 1.452.1.421:1
422. Open CASCADE STEP translator 6.8 1.452.1.422:1
423. Open CASCADE STEP translator 6.8 1.452.1.423:1
424. Open CASCADE STEP translator 6.8 1.452.1.424:1
425. Open CASCADE STEP translator 6.8 1.452.1.425:1
426. Open CASCADE STEP translator 6.8 1.452.1.426:1
427. Open CASCADE STEP translator 6.8 1.452.1.427:1
428. Open CASCADE STEP translator 6.8 1.452.1.428:1
429. Open CASCADE STEP translator 6.8 1.452.1.429:1
430. Open CASCADE STEP translator 6.8 1.452.1.430:1
431. Open CASCADE STEP translator 6.8 1.452.1.431:1
432. Open CASCADE STEP translator 6.8 1.452.1.432:1
433. Open CASCADE STEP translator 6.8 1.452.1.433:1
434. Open CASCADE STEP translator 6.8 1.452.1.434:1
435. Open CASCADE STEP translator 6.8 1.452.1.435:1
436. Open CASCADE STEP translator 6.8 1.452.1.436:1
437. Open CASCADE STEP translator 6.8 1.452.1.437:1
438. Open CASCADE STEP translator 6.8 1.452.1.438:1
439. Open CASCADE STEP translator 6.8 1.452.1.439:1
440. Open CASCADE STEP translator 6.8 1.452.1.440:1
441. Open CASCADE STEP translator 6.8 1.452.1.441:1
442. Open CASCADE STEP translator 6.8 1.452.1.442:1
443. Open CASCADE STEP translator 6.8 1.452.1.443:1
444. Open CASCADE STEP translator 6.8 1.452.1.444:1
445. Open CASCADE STEP translator 6.8 1.452.1.445:1
446. Open CASCADE STEP translator 6.8 1.452.1.446:1
447. Open CASCADE STEP translator 6.8 1.452.1.447:1
448. Open CASCADE STEP translator 6.8 1.452.1.448:1
449. Open CASCADE STEP translator 6.8 1.452.1.449:1
450. Open CASCADE STEP translator 6.8 1.452.1.450:1
451. Open CASCADE STEP translator 6.8 1.452.1.451:1
452. Open CASCADE STEP translator 6.8 1.452.1.452:1
453. Open CASCADE STEP translator 6.8 1.452.1.453:1
454. Open CASCADE STEP translator 6.8 1.452.1.454:1
455. Open CASCADE STEP translator 6.8 1.452.1.455:1
456. Open CASCADE STEP translator 6.8 1.452.1.456:1
457. Open CASCADE STEP translator 6.8 1.452.1.457:1
458. Open CASCADE STEP translator 6.8 1.452.1.458:1
459. Open CASCADE STEP translator 6.8 1.452.1.459:1
460. Open CASCADE STEP translator 6.8 1.452.1.460:1
461. Open CASCADE STEP translator 6.8 1.452.1.461:1
462. Open CASCADE STEP translator 6.8 1.452.1.462:1
463. Open CASCADE STEP translator 6.8 1.452.1.463:1
464. Open CASCADE STEP translator 6.8 1.452.1.464:1
465. Open CASCADE STEP translator 6.8 1.452.1.465:1
466. Open CASCADE STEP translator 6.8 1.452.1.466:1
467. Open CASCADE STEP translator 6.8 1.452.1.467:1
468. Open CASCADE STEP translator 6.8 1.452.1.468:1
469. Open CASCADE STEP translator 6.8 1.452.1.469:1
470. Open CASCADE STEP translator 6.8 1.452.1.470:1
471. Open CASCADE STEP translator 6.8 1.452.1.471:1
472. Open CASCADE STEP translator 6.8 1.452.1.472:1
473. Open CASCADE STEP translator 6.8 1.452.1.473:1
474. Open CASCADE STEP translator 6.8 1.452.1.474:1
475. Open CASCADE STEP translator 6.8 1.452.1.475:1
476. Open CASCADE STEP translator 6.8 1.452.1.476:1
477. Open CASCADE STEP translator 6.8 1.452.1.477:1
478. Open CASCADE STEP translator 6.8 1.452.1.478:1
479. Open CASCADE STEP translator 6.8 1.452.1.479:1
480. Open CASCADE STEP translator 6.8 1.452.1.480:1
481. Open CASCADE STEP translator 6.8 1.452.1.481:1
482. Open CASCADE STEP translator 6.8 1.452.1.482:1
483. Open CASCADE STEP translator 6.8 1.452.1.483:1
484. Open CASCADE STEP translator 6.8 1.452.1.484:1
485. Open CASCADE STEP translator 6.8 1.452.1.485:1
486. Open CASCADE STEP translator 6.8 1.452.1.486:1
487. Open CASCADE STEP translator 6.8 1.452.1.487:1
488. Open CASCADE STEP translator 6.8 1.452.1.488:1
489. Open CASCADE STEP translator 6.8 1.452.1.489:1
490. Open CASCADE STEP translator 6.8 1.452.1.490:1
491. Open CASCADE STEP translator 6.8 1.452.1.491:1
492. Open CASCADE STEP translator 6.8 1.452.1.492:1
493. Open CASCADE STEP translator 6.8 1.452.1.493:1
494. Open CASCADE STEP translator 6.8 1.452.1.494:1
495. Open CASCADE STEP translator 6.8 1.452.1.495:1
496. Open CASCADE STEP translator 6.8 1.452.1.496:1
497. Open CASCADE STEP translator 6.8 1.452.1.497:1
498. Open CASCADE STEP translator 6.8 1.452.1.498:1
499. Open CASCADE STEP translator 6.8 1.452.1.499:1
500. Open CASCADE STEP translator 6.8 1.452.1.500:1
501. Open CASCADE STEP translator 6.8 1.452.1.501:1
502. Open CASCADE STEP translator 6.8 1.452.1.502:1
503. Open CASCADE STEP translator 6.8 1.452.1.503:1
504. Open CASCADE STEP translator 6.8 1.452.1.504:1
505. Open CASCADE STEP translator 6.8 1.452.1.505:1
506. Open CASCADE STEP translator 6.8 1.452.1.506:1
507. Open CASCADE STEP translator 6.8 1.452.1.507:1
508. Open CASCADE STEP translator 6.8 1.452.1.508:1
509. Open CASCADE STEP translator 6.8 1.452.1.509:1
510. Open CASCADE STEP translator 6.8 1.452.1.510:1
511. Open CASCADE STEP translator 6.8 1.452.1.511:1
512. Open CASCADE STEP translator 6.8 1.452.1.512:1
513. Open CASCADE STEP translator 6.8 1.452.1.513:1
514. Open CASCADE STEP translator 6.8 1.452.1.514:1
515. Open CASCADE STEP translator 6.8 1.452.1.515:1
516. Open CASCADE STEP translator 6.8 1.452.1.516:1
517. Open CASCADE STEP translator 6.8 1.452.1.517:1
518. Open CASCADE STEP translator 6.8 1.452.1.518:1
519. Open CASCADE STEP translator 6.8 1.452.1.519:1
520. Open CASCADE STEP translator 6.8 1.452.1.520:1
521. Open CASCADE STEP translator 6.8 1.452.1.521:1
522. Open CASCADE STEP translator 6.8 1.452.1.522:1
523. Open CASCADE STEP translator 6.8 1.452.1.523:1
524. Open CASCADE STEP translator 6.8 1.452.1.524:1
525. Open CASCADE STEP translator 6.8 1.452.1.525:1
526. Open CASCADE STEP translator 6.8 1.452.1.526:1
527. Open CASCADE STEP translator 6.8 1.452.1.527:1
528. Open CASCADE STEP translator 6.8 1.452.1.528:1
529. Open CASCADE STEP translator 6.8 1.452.1.529:1
530. Open CASCADE STEP translator 6.8 1.452.1.530:1
531. Open CASCADE STEP translator 6.8 1.452.1.531:1
532. Open CASCADE STEP translator 6.8 1.452.1.532:1
533. Open CASCADE STEP translator 6.8 1.452.1.533:1
534. Open CASCADE STEP translator 6.8 1.452.1.534:1
535. Open CASCADE STEP translator 6.8 1.452.1.535:1
536. Open CASCADE STEP translator 6.8 1.452.1.536:1
537. Open CASCADE STEP translator 6.8 1.452.1.537:1
538. Open CASCADE STEP translator 6.8 1.452.1.538:1
539. Open CASCADE STEP translator 6.8 1.452.1.539:1
540. Open CASCADE STEP translator 6.8 1.452.1.540:1
541. Open CASCADE STEP translator 6.8 1.452.1.541:1
542. Open CASCADE STEP translator 6.8 1.452.1.542:1
543. Open CASCADE STEP translator 6.8 1.452.1.543:1
544. Open CASCADE STEP translator 6.8 1.452.1.544:1
545. Open CASCADE STEP translator 6.8 1.452.1.545:1
546. Open CASCADE STEP translator 6.8 1.452.1.546:1
547. Open CASCADE STEP translator 6.8 1.452.1.547:1
548. Open CASCADE STEP translator 6.8 1.452.1.548:1
549. Open CASCADE STEP translator 6.8 1.452.1.549:1
550. Open CASCADE STEP translator 6.8 1.452.1.550:1
551. Open CASCADE STEP translator 6.8 1.452.1.551:1
552. Open CASCADE STEP translator 6.8 1.452.1.552:1
553. Open CASCADE STEP translator 6.8 1.452.1.553:1
554. Open CASCADE STEP translator 6.8 1.452.1.554:1
555. Open CASCADE STEP translator 6.8 1.452.1.555:1
556. Open CASCADE STEP translator 6.8 1.452.1.556:1
557. Open CASCADE STEP translator 6.8 1.452.1.557:1
558. Open CASCADE STEP translator 6.8 1.452.1.558:1
559. Open CASCADE STEP translator 6.8 1.452.1.559:1
560. Open CASCADE STEP translator 6.8 1.452.1.560:1
561. Open CASCADE STEP translator 6.8 1.452.1.561:1
562. Open CASCADE STEP translator 6.8 1.452.1.562:1
563. Open CASCADE STEP translator 6.8 1.452.1.563:1
564. Open CASCADE STEP translator 6.8 1.452.1.564:1
565. Open CASCADE STEP translator 6.8 1.452.1.565:1
566. Open CASCADE STEP translator 6.8 1.452.1.566:1
567. Open CASCADE STEP translator 6.8 1.452.1.567:1
568. Open CASCADE STEP translator 6.8 1.452.1.568:1
569. Open CASCADE STEP translator 6.8 1.452.1.569:1
570. Open CASCADE STEP translator 6.8 1.452.1.570:1
571. Open CASCADE STEP translator 6.8 1.452.1.571:1
572. Open CASCADE STEP translator 6.8 1.452.1.572:1
573. Open CASCADE STEP translator 6.8 1.452.1.573:1
574. Open CASCADE STEP translator 6.8 1.452.1.574:1
575. Open CASCADE STEP translator 6.8 1.452.1.575:1
576. Open CASCADE STEP translator 6.8 1.452.1.576:1
577. Open CASCADE STEP translator 6.8 1.452.1.577:1
578. Open CASCADE STEP translator 6.8 1.452.1.578:1
579. Open CASCADE STEP translator 6.8 1.452.1.579:1
580. Open CASCADE STEP translator 6.8 1.452.1.580:1
581. Open CASCADE STEP translator 6.8 1.452.1.581:1
582. Open CASCADE STEP translator 6.8 1.452.1.582:1
583. Open CASCADE STEP translator 6.8 1.452.1.583:1
584. Open CASCADE STEP translator 6.8 1.452.1.584:1
585. Open CASCADE STEP translator 6.8 1.452.1.585:1
586. Open CASCADE STEP translator 6.8 1.452.1.586:1
587. Open CASCADE STEP translator 6.8 1.452.1.587:1
588. Open CASCADE STEP translator 6.8 1.452.1.588:1
589. Open CASCADE STEP translator 6.8 1.452.1.589:1
590. Open CASCADE STEP translator 6.8 1.452.1.590:1
591. Open CASCADE STEP translator 6.8 1.452.1.591:1